# Autodesk Inventor assembly: Assieme 2 - Taglio
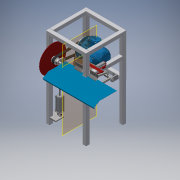
[picture p0: Inventor's stored thumbnail of the model, 180x180]
Saved by Autodesk Inventor 2018 (Build 220112000, 112)
## iProperties
Created: 2020-06-01
Part Number: Assieme 2 - Taglio
Material: Generico
Document SubType Name: Weldment
Designer: Francesco
Weld Material: Welded Aluminum-6061
Author: Francesco
## Documents named in this file (13)
- C:\Users\Francesco\no-brim\Meccanica\Progetto Inventor no-brim\Assiemi\Assieme 2 - Taglio.iam
- C:\Users\Francesco\no-brim\Meccanica\Progetto Inventor no-brim\Assiemi\Telaio - Taglio.iam
- C:\Users\Francesco\no-brim\Meccanica\Progetto Inventor no-brim\Assiemi\Trasmissione cinghie - Taglio.iam
- C:\Users\Francesco\no-brim\Meccanica\Progetto Inventor no-brim\Unificati\it-IT\SKF B - angular contact\SKF B7202 BE.ipt
- C:\Users\Francesco\no-brim\Meccanica\Progetto Inventor no-brim\Parti\Porta cuscinetto perno telaietto.ipt
- C:\Users\Francesco\no-brim\Meccanica\Progetto Inventor no-brim\Parti\Forcella movimento lama 2.ipt
- C:\Users\Francesco\no-brim\Meccanica\Progetto Inventor no-brim\Parti\Perno forcella.ipt
- C:\Users\Francesco\no-brim\Meccanica\Progetto Inventor no-brim\Parti\Pistone salita lama d 40 c 100\AIS2017\536288 ADN-40-100-I-P-A---(0).iam
- C:\Users\Francesco\no-brim\Meccanica\Progetto Inventor no-brim\Parti\Piano lamiera scarico.ipt
- C:\Users\Francesco\no-brim\Meccanica\Progetto Inventor no-brim\Assiemi\Pistone scarico - Taglio.iam
- C:\Users\Francesco\no-brim\Meccanica\Progetto Inventor no-brim\Parti\Piastra supporto pistone lama.ipt
- C:\Users\Francesco\no-brim\Meccanica\Progetto Inventor no-brim\Parti\Forcella movimento lama 3.ipt
- C:\Users\Francesco\no-brim\Meccanica\Progetto Inventor no-brim\Parti\Supporto salita lama.ipt
## Components (17 placed, 11 different names)
1. Telaio - Taglio:1 [sub-assembly] — Coincidente:5, Coincidente:7, Allineato:1, Allineato:3, Coincidente:22, Allineato:14, Coincidente:23, Coincidente:24, Coincidente:25, Coincidente:26, Allineato:16, Coincidente:63, Coincidente:64
2. Trasmissione cinghie - Taglio:2 [sub-assembly] — Coincidente:9, Allineato:11, Angolo:12, Coincidente:60, Coincidente:61
3. SKF B- Contatto angolare SKF B7202 BE:1 — Coincidente:1, Coincidente:4, Coincidente:9
4. SKF B- Contatto angolare SKF B7202 BE:2 — Coincidente:2, Coincidente:3
5. Porta cuscinetto perno telaietto:1 — Coincidente:2, Coincidente:3, Coincidente:7, Allineato:2
6. Porta cuscinetto perno telaietto:2 — Coincidente:1, Coincidente:4, Coincidente:5, Allineato:1, Allineato:2, Allineato:16
7. Piano lamiera scarico:1 — Coincidente:22, Allineato:14, Coincidente:23
8. Pistone scarico - Taglio:1 [sub-assembly] — Coincidente:24, Coincidente:25, Coincidente:26
9. 536288 ADN-40-100-I-P-A---(0):2 [sub-assembly] — Coincidente:42, Angolo:6, Coincidente:43, Coincidente:52, Coincidente:53, Angolo:8
10. Piastra supporto pistone lama:1 — Coincidente:42, Angolo:6, Coincidente:43, Coincidente:48, Coincidente:49, Angolo:7
11. Perno forcella:2 — Coincidente:47, Allineato:18, Coincidente:50, Allineato:19
12. Forcella movimento lama:5 — Coincidente:47, Coincidente:48, Allineato:18, Coincidente:49, Angolo:7
13. Forcella movimento lama:6 — Coincidente:50, Allineato:19, Coincidente:62
14. Forcella movimento lama:7 — Coincidente:52, Coincidente:53, Angolo:8, Coincidente:54, Allineato:20
15. Perno forcella:3 — Coincidente:51, Coincidente:54, Allineato:20, Coincidente:55, Allineato:21
16. Forcella movimento lama:10 — Coincidente:51, Coincidente:55, Allineato:21, Angolo:12, Coincidente:60, Coincidente:61
17. Supporto salita lama:1 — Coincidente:62, Coincidente:63, Coincidente:64
## Relationships (42: Mate 28, Flush 10, Angle 4)
- Coincidente:1 [Mate]: SKF B- Contatto angolare SKF B7202 BE:1 ↔ Porta cuscinetto perno telaietto:2
- Coincidente:2 [Mate]: SKF B- Contatto angolare SKF B7202 BE:2 ↔ Porta cuscinetto perno telaietto:1
- Coincidente:3 [Mate]: SKF B- Contatto angolare SKF B7202 BE:2 ↔ Porta cuscinetto perno telaietto:1
- Coincidente:4 [Mate]: SKF B- Contatto angolare SKF B7202 BE:1 ↔ Porta cuscinetto perno telaietto:2
- Coincidente:5 [Mate]: Telaio - Taglio:1 ↔ Porta cuscinetto perno telaietto:2
- Coincidente:7 [Mate]: Telaio - Taglio:1 ↔ Porta cuscinetto perno telaietto:1
- Allineato:1 [Flush] (-2.5 mm): Telaio - Taglio:1 ↔ Porta cuscinetto perno telaietto:2
- Allineato:2 [Flush]: Porta cuscinetto perno telaietto:1 ↔ Porta cuscinetto perno telaietto:2
- Coincidente:9 [Mate]: Trasmissione cinghie - Taglio:2 ↔ SKF B- Contatto angolare SKF B7202 BE:1
- Allineato:3 [Flush] (-225 mm): Telaio - Taglio:1
- Allineato:11 [Flush]: Trasmissione cinghie - Taglio:2
- Coincidente:22 [Mate]: Telaio - Taglio:1 ↔ Piano lamiera scarico:1
- Allineato:14 [Flush]: Telaio - Taglio:1 ↔ Piano lamiera scarico:1
- Coincidente:23 [Mate] (2.5 mm): Telaio - Taglio:1 ↔ Piano lamiera scarico:1
- Coincidente:24 [Mate]: Telaio - Taglio:1 ↔ Pistone scarico - Taglio:1
- Coincidente:25 [Mate] (0.5 mm): Telaio - Taglio:1 ↔ Pistone scarico - Taglio:1
- Coincidente:26 [Mate] (185 mm): Telaio - Taglio:1 ↔ Pistone scarico - Taglio:1
- Allineato:16 [Flush] (55 mm): Telaio - Taglio:1 ↔ Porta cuscinetto perno telaietto:2
- Coincidente:42 [Mate]: 536288 ADN-40-100-I-P-A---(0):2 ↔ Piastra supporto pistone lama:1
- Angolo:6 [Angle] (0 deg): 536288 ADN-40-100-I-P-A---(0):2 ↔ Piastra supporto pistone lama:1
- Coincidente:43 [Mate]: 536288 ADN-40-100-I-P-A---(0):2 ↔ Piastra supporto pistone lama:1
- Coincidente:47 [Mate]: Perno forcella:2 ↔ Forcella movimento lama:5
- Coincidente:48 [Mate]: Piastra supporto pistone lama:1 ↔ Forcella movimento lama:5
- Allineato:18 [Flush] (-11 mm): Perno forcella:2 ↔ Forcella movimento lama:5
- Coincidente:49 [Mate]: Piastra supporto pistone lama:1 ↔ Forcella movimento lama:5
- Angolo:7 [Angle] (0 deg): Piastra supporto pistone lama:1 ↔ Forcella movimento lama:5
- Coincidente:50 [Mate]: Perno forcella:2 ↔ Forcella movimento lama:6
- Allineato:19 [Flush] (2.5 mm): Perno forcella:2 ↔ Forcella movimento lama:6
- Coincidente:51 [Mate]: Perno forcella:3 ↔ Forcella movimento lama:10
- Coincidente:52 [Mate]: 536288 ADN-40-100-I-P-A---(0):2 ↔ Forcella movimento lama:7
- Coincidente:53 [Mate]: 536288 ADN-40-100-I-P-A---(0):2 ↔ Forcella movimento lama:7
- Angolo:8 [Angle] (0 deg): 536288 ADN-40-100-I-P-A---(0):2 ↔ Forcella movimento lama:7
- Coincidente:54 [Mate]: Forcella movimento lama:7 ↔ Perno forcella:3
- Allineato:20 [Flush] (-11 mm): Forcella movimento lama:7 ↔ Perno forcella:3
- Coincidente:55 [Mate]: Perno forcella:3 ↔ Forcella movimento lama:10
- Allineato:21 [Flush] (2.5 mm): Perno forcella:3 ↔ Forcella movimento lama:10
- Angolo:12 [Angle] (0 deg): Trasmissione cinghie - Taglio:2 ↔ Forcella movimento lama:10
- Coincidente:60 [Mate]: Trasmissione cinghie - Taglio:2 ↔ Forcella movimento lama:10
- Coincidente:61 [Mate]: Trasmissione cinghie - Taglio:2 ↔ Forcella movimento lama:10
- Coincidente:62 [Mate]: Forcella movimento lama:6 ↔ Supporto salita lama:1
- Coincidente:63 [Mate]: Telaio - Taglio:1 ↔ Supporto salita lama:1
- Coincidente:64 [Mate]: Telaio - Taglio:1 ↔ Supporto salita lama:1
